# Autodesk Inventor assembly: lcd_controller
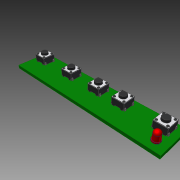
[picture p0: Inventor's stored thumbnail of the model, 180x180]
Saved by Autodesk Inventor 2014 (Build 180170000, 170)
## iProperties
Created: 2014-03-23
Part Number: lcd_controller
Document SubType Name: Assembly
Designer: buben
Author: buben
## Documents named in this file (4)
- C:\Users\buben\Documents\GitHub\bacon\inventor files\utils\main_lcd_controller\lcd_controller.iam
- C:\Users\buben\Documents\GitHub\bacon\inventor files\utils\main_lcd_controller\lcd_controller_pcb.ipt
- C:\Users\buben\Documents\GitHub\bacon\inventor files\3rd party components\tactileswitch-short\Imported Components\tactileswitch-short\tactileswitch-short.ipt
- C:\Users\buben\Documents\GitHub\bacon\inventor files\3rd party components\led_3mm_red\Imported Components\LED 3mm RED\LED 3mm RED.ipt
## Components (7 placed, 3 different names)
1. lcd_controller_pcb:1 — Mate:1, Mate:2, Mate:3, Mate:4, Mate:5, Mate:8, Mate:9, Mate:10, Flush:5, Flush:6, Mate:15, Mate:16, Angle:1, Mate:17
2. tactileswitch-short:1 — Mate:5, Flush:1, Mate:11
3. tactileswitch-short:2 — Mate:4, Flush:1, Flush:2, Mate:11, Mate:12
4. tactileswitch-short:3 — Mate:3, Flush:2, Flush:3, Mate:12, Mate:13
5. tactileswitch-short:4 — Mate:2, Flush:3, Flush:4, Mate:13, Mate:14
6. tactileswitch-short:5 — Mate:1, Flush:4, Mate:14, Flush:5, Flush:6
7. LED 3mm RED:1 — Mate:15, Mate:16, Angle:1, Mate:17
## Relationships (22: Mate 15, Flush 6, Angle 1)
- Mate:1: lcd_controller_pcb:1 ↔ tactileswitch-short:5
- Mate:2: lcd_controller_pcb:1 ↔ tactileswitch-short:4
- Mate:3: lcd_controller_pcb:1 ↔ tactileswitch-short:3
- Mate:4: lcd_controller_pcb:1 ↔ tactileswitch-short:2
- Mate:5: lcd_controller_pcb:1 ↔ tactileswitch-short:1
- Flush:1: tactileswitch-short:1 ↔ tactileswitch-short:2
- Flush:2: tactileswitch-short:2 ↔ tactileswitch-short:3
- Flush:3: tactileswitch-short:3 ↔ tactileswitch-short:4
- Flush:4: tactileswitch-short:4 ↔ tactileswitch-short:5
- Mate:8: lcd_controller_pcb:1
- Mate:9: lcd_controller_pcb:1
- Mate:10: lcd_controller_pcb:1
- Mate:11 (12.25 mm): tactileswitch-short:1 ↔ tactileswitch-short:2
- Mate:12 (9.8 mm): tactileswitch-short:2 ↔ tactileswitch-short:3
- Mate:13 (6.4 mm): tactileswitch-short:3 ↔ tactileswitch-short:4
- Mate:14 (12 mm): tactileswitch-short:4 ↔ tactileswitch-short:5
- Flush:5 (-2 mm): lcd_controller_pcb:1 ↔ tactileswitch-short:5
- Flush:6 (-3 mm): lcd_controller_pcb:1 ↔ tactileswitch-short:5
- Mate:15 (1 mm): lcd_controller_pcb:1 ↔ LED 3mm RED:1
- Mate:16 (-4.2 mm): lcd_controller_pcb:1 ↔ LED 3mm RED:1
- Angle:1 (0 deg): lcd_controller_pcb:1 ↔ LED 3mm RED:1
- Mate:17 (-3.5 mm): lcd_controller_pcb:1 ↔ LED 3mm RED:1
